# Autodesk Inventor assembly: mesa_aquecimento
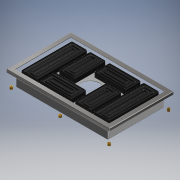
[picture p0: Inventor's stored thumbnail of the model, 180x180]
Saved by Autodesk Inventor 2018 (Build 220112000, 112)
## iProperties
Created: 2018-05-03
Part Number: mesa_aquecimento
Material: Genérico
Document SubType Name: Assembly
Designer: Georgines
Author: Georgines
## Documents named in this file (8)
- C:\Users\Georgines\Downloads\pecas_3d-20180530T120808Z-001\pecas_3d\mesa_aquecimento.iam
- C:\Users\Georgines\Downloads\pecas_3d-20180530T120808Z-001\pecas_3d\resistencia_original_2.ipt
- C:\Users\Georgines\Downloads\pecas_3d-20180530T120808Z-001\pecas_3d\resistencia_600w.ipt
- C:\Users\Georgines\Downloads\pecas_3d-20180530T120808Z-001\pecas_3d\base_interna_resistencias.ipt
- C:\Users\Georgines\Downloads\pecas_3d-20180530T120808Z-001\pecas_3d\base_externa_resistencias.ipt
- C:\Users\Georgines\Downloads\pecas_3d-20180530T120808Z-001\pecas_3d\tampa_superior_resistencias.ipt
- C:\Users\Georgines\Downloads\pecas_3d-20180530T120808Z-001\pecas_3d\espassador_mesa_resistencias.ipt
- C:\Users\Georgines\Downloads\pecas_3d-20180530T120808Z-001\pecas_3d\chapa_referencia_tampa_gabinete.ipt
## Components (16 placed, 7 different names)
1. resistencia_original_2:2 — Coincidência:2, Alinhamento:5, Coincidência:4, Alinhamento:7, Alinhamento:8, Alinhamento:11, Coincidência:7
2. resistencia_original_2:3 — Coincidência:1, Alinhamento:1, Alinhamento:2, Coincidência:3, Alinhamento:6, Coincidência:5, Alinhamento:9, Alinhamento:10, Coincidência:6, Alinhamento:14, Alinhamento:15
3. resistencia_original_2:1 — Coincidência:1, Alinhamento:1, Alinhamento:2, Coincidência:2, Alinhamento:5, Alinhamento:8, Alinhamento:9, Alinhamento:13, Alinhamento:16
4. resistencia_original_2:4 — Coincidência:3, Alinhamento:6, Coincidência:4, Alinhamento:7, Coincidência:5, Alinhamento:10, Alinhamento:11
5. resistencia_600w:1 — Coincidência:6, Alinhamento:14, Alinhamento:15, Alinhamento:17
6. resistencia_600w:2 — Coincidência:7, Alinhamento:13, Alinhamento:16
7. base_interna_resistencias:1 — Alinhamento:17, Alinhamento:18
8. base_externa_resistencias:1 — Alinhamento:18, Alinhamento:19, Alinhamento:20, Inserir:1, Inserir:2, Inserir:3, Inserir:4, Inserir:5, Alinhamento:21
9. tampa_superior_resistencias:1 — Alinhamento:19
10. espassador_mesa_resistencias — Alinhamento:20
11. espassador_mesa_resistencias:1 — Inserir:4
12. espassador_mesa_resistencias:2 — Inserir:1
13. espassador_mesa_resistencias:3 — Inserir:2
14. espassador_mesa_resistencias:4 — Inserir:3
15. espassador_mesa_resistencias:5 — Inserir:5
16. chapa_referencia_tampa_gabinete:1 — Alinhamento:22
## Relationships (31: Flush 19, Mate 7, Insert 5)
- Coincidência:1 [Mate] (14 mm): resistencia_original_2:3 ↔ resistencia_original_2:1
- Alinhamento:1 [Flush]: resistencia_original_2:3 ↔ resistencia_original_2:1
- Alinhamento:2 [Flush]: resistencia_original_2:3 ↔ resistencia_original_2:1
- Coincidência:2 [Mate] (14 mm): resistencia_original_2:2 ↔ resistencia_original_2:1
- Alinhamento:5 [Flush]: resistencia_original_2:2 ↔ resistencia_original_2:1
- Coincidência:3 [Mate] (14 mm): resistencia_original_2:3 ↔ resistencia_original_2:4
- Alinhamento:6 [Flush]: resistencia_original_2:3 ↔ resistencia_original_2:4
- Coincidência:4 [Mate] (14 mm): resistencia_original_2:2 ↔ resistencia_original_2:4
- Alinhamento:7 [Flush]: resistencia_original_2:2 ↔ resistencia_original_2:4
- Coincidência:5 [Mate] (14 mm): resistencia_original_2:3 ↔ resistencia_original_2:4
- Alinhamento:8 [Flush]: resistencia_original_2:2 ↔ resistencia_original_2:1
- Alinhamento:9 [Flush]: resistencia_original_2:3 ↔ resistencia_original_2:1
- Alinhamento:10 [Flush]: resistencia_original_2:3 ↔ resistencia_original_2:4
- Alinhamento:11 [Flush]: resistencia_original_2:2 ↔ resistencia_original_2:4
- Coincidência:6 [Mate] (10 mm): resistencia_original_2:3 ↔ resistencia_600w:1
- Coincidência:7 [Mate] (10 mm): resistencia_original_2:2 ↔ resistencia_600w:2
- Alinhamento:13 [Flush]: resistencia_original_2:1 ↔ resistencia_600w:2
- Alinhamento:14 [Flush]: resistencia_original_2:3 ↔ resistencia_600w:1
- Alinhamento:15 [Flush]: resistencia_original_2:3 ↔ resistencia_600w:1
- Alinhamento:16 [Flush]: resistencia_original_2:1 ↔ resistencia_600w:2
- Alinhamento:17 [Flush]: resistencia_600w:1 ↔ base_interna_resistencias:1
- Alinhamento:18 [Flush]: base_interna_resistencias:1 ↔ base_externa_resistencias:1
- Alinhamento:19 [Flush]: base_externa_resistencias:1 ↔ tampa_superior_resistencias:1
- Alinhamento:20 [Flush]: base_externa_resistencias:1 ↔ espassador_mesa_resistencias
- Inserir:1: base_externa_resistencias:1 ↔ espassador_mesa_resistencias:2
- Inserir:2: base_externa_resistencias:1 ↔ espassador_mesa_resistencias:3
- Inserir:3: base_externa_resistencias:1 ↔ espassador_mesa_resistencias:4
- Inserir:4: base_externa_resistencias:1 ↔ espassador_mesa_resistencias:1
- Inserir:5: base_externa_resistencias:1 ↔ espassador_mesa_resistencias:5
- Alinhamento:21 [Flush] (8 mm): base_externa_resistencias:1
- Alinhamento:22 [Flush]: chapa_referencia_tampa_gabinete:1
